# Autodesk Inventor assembly: Sessao_28_03_001_001
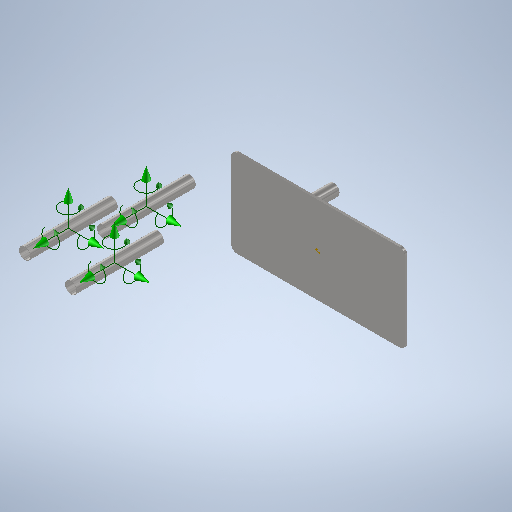
[picture p0: Inventor's stored thumbnail of the model, 512x512]
Saved by Autodesk Inventor 2026 (Build 300175000, 175)
## iProperties
Created: 2025-03-28
Part Number: Sessao_28_03_001_001
Document SubType Name: Assembly
Designer: Carlos Dias
Author: Carlos Dias
## Documents named in this file (3)
- C:\Users\Carlos Dias\Documents\Formação-TEARCI\UFCDs\5134 - Robótica _ Fundamentos\Material De Apoio\Sessao_28_03\Sessao_28_03_001_001.iam
- C:\Users\Carlos Dias\Documents\Formação-TEARCI\UFCDs\5134 - Robótica _ Fundamentos\Material De Apoio\Sessao_28_03\Sessao_28_03_001_001.ipt
- C:\Users\Carlos Dias\Documents\Formação-TEARCI\UFCDs\5134 - Robótica _ Fundamentos\Material De Apoio\Sessao_28_03\Sessao_28_03_002_001.ipt
## Components (5 placed, 2 different names)
1. Sessao_28_03_001_001:1 — Flush:1, Flush:2, Flush:3, Mate:1
2. Sessao_28_03_002_001:1
3. Sessao_28_03_002_001:2
4. Sessao_28_03_002_001:3
5. Sessao_28_03_002_001:4 — Mate:1, Flush:4, Flush:5
## Relationships (6: Flush 5, Mate 1)
- Flush:1: Sessao_28_03_001_001:1
- Flush:2: Sessao_28_03_001_001:1
- Flush:3: Sessao_28_03_001_001:1
- Mate:1: Sessao_28_03_001_001:1 ↔ Sessao_28_03_002_001:4
- Flush:4 (635 mm): Sessao_28_03_002_001:4
- Flush:5 (250 mm): Sessao_28_03_002_001:4
